# Autodesk Inventor assembly: walls
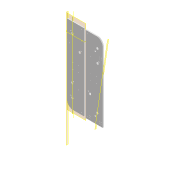
[picture p0: Inventor's stored thumbnail of the model, 180x180]
Saved by Autodesk Inventor 2020 (Build 240168000, 168)
## iProperties
Created: 2019-11-20
Part Number: walls
Document SubType Name: Assembly
Designer: ball
Author: ball
## Documents named in this file (3)
- C:\FTC\FTC8863CAD\2019 Robot\Mecanum Drive Train\walls.iam
- C:\FTC\FTC8863CAD\2019 Robot\Mecanum Drive Train\outside wall test.ipt
- C:\FTC\FTC8863CAD\2019 Robot\Mecanum Drive Train\inside wall test.ipt
## Components (2 placed, 2 different names)
1. outside wall test:1 — Mate:1, Flush:1
2. inside wall test:1 — Mate:2, Flush:1
## Relationships (3: Mate 2, Flush 1)
- Mate:1: outside wall test:1
- Mate:2 (114.3 mm): inside wall test:1
- Flush:1: outside wall test:1 ↔ inside wall test:1
